# Autodesk Inventor assembly: V5H1
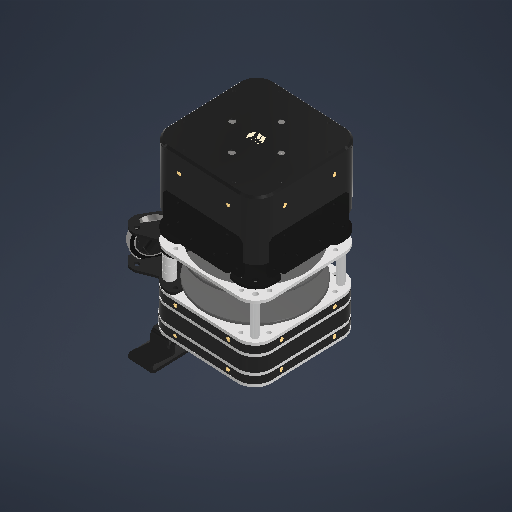
[picture p0: Inventor's stored thumbnail of the model, 512x512]
Saved by Autodesk Inventor 2026.1 (Build 301233000, 233)
## iProperties
Created: 2026-05-18
Part Number: V5H1
Document SubType Name: Assembly
Designer: aaron
Author: aaron
## Documents named in this file (18)
- D:\work\loopandpixel\openworkoutsystem\cad\v5\V5H1.iam
- D:\work\loopandpixel\openworkoutsystem\cad\v5\motor.iam
- D:\work\loopandpixel\openworkoutsystem\cad\v5\handle_metal.ipt
- D:\work\loopandpixel\openworkoutsystem\cad\v5\handle_insert.ipt
- D:\work\loopandpixel\openworkoutsystem\cad\v5\spool.iam
- D:\work\loopandpixel\openworkoutsystem\cad\v5\output_support.ipt
- D:\work\loopandpixel\openworkoutsystem\cad\v5\spool_spacer_driver.ipt
- D:\work\loopandpixel\openworkoutsystem\cad\v5\spool_spacer.ipt
- D:\work\loopandpixel\openworkoutsystem\cad\v5\M5x40mm_coupler.ipt
- D:\work\loopandpixel\openworkoutsystem\cad\v5\bearings\bearing_42x30x7.ipt
- D:\work\loopandpixel\openworkoutsystem\cad\v5\head_innter_top_42.ipt
- D:\work\loopandpixel\openworkoutsystem\cad\v5\bearings\bearing_12x8x8.ipt
- D:\work\loopandpixel\openworkoutsystem\cad\v5\stator_center_00_alu.ipt
- D:\work\loopandpixel\openworkoutsystem\cad\v5\moteus\20250427-moteus-x1-r1\20250427-moteus-x1-r1\20250427-moteus-x1-r1.ipt
- D:\work\loopandpixel\openworkoutsystem\cad\v5\20250328-x1-heat-spreader\20250328-x1-heat-spreader\20250328-x1-heat-spreader.ipt
- D:\work\loopandpixel\openworkoutsystem\cad\v5\mcthermal_plate.ipt
- D:\work\loopandpixel\openworkoutsystem\cad\v5\battery_pack_16s.ipt.iam
- battery_pack_16s.ipt
## Components (25 placed, 16 different names)
1. motor:1 [sub-assembly] — Insert:1, Insert:2, Insert:5, Insert:6, Insert:12, Insert:13
2. handle_metal:1 — Insert:1, Insert:2, Insert:3, Insert:4
3. handle_insert:1 — Insert:3, Insert:4
4. spool:1 [sub-assembly] — Insert:10, Insert:11
5. output_support:1 — Insert:16, Insert:19
6. output_support:2 — Insert:12, Insert:13, Mate:1, Insert:28, Insert:29
7. spool_spacer_driver:2 — Insert:6
8. spool_spacer_driver:3 — Insert:5, Insert:9
9. spool_spacer:1 — Insert:9, Insert:10
10. spool_spacer:2 — Insert:11
11. M5x40mm_coupler:1 — Insert:16, Insert:24, Insert:29
12. M5x40mm_coupler:2 — Insert:19, Mate:2, Insert:27, Insert:28
13. M5x40mm_coupler:3 — Insert:25
14. M5x40mm_coupler:4 — Insert:26
15. bearing_42x30x7:1 — Insert:20, Mate:1
16. head_innter_top_42:1 — Insert:20
17. bearing_12x8x8:1 — Mate:2, Insert:21
18. bearing_12x8x8:2 — Insert:21, Insert:22
19. bearing_12x8x8:3 — Insert:22, Insert:23
20. bearing_12x8x8:4 — Insert:23
21. stator_center_00_alu:1 — Insert:24, Insert:25, Insert:26, Insert:27, Flush:3, Flush:4
22. 20250427-moteus-x1-r1:1
23. 20250328-x1-heat-spreader:1
24. mcthermal_plate:1
25. battery_pack_16s.ipt:1 [sub-assembly] — Flush:3, Flush:4
## Relationships (35: Insert 27, Mate 4, Flush 4)
- Insert:1: motor:1 ↔ handle_metal:1
- Insert:2: motor:1 ↔ handle_metal:1
- Insert:3: handle_metal:1 ↔ handle_insert:1
- Insert:4: handle_metal:1 ↔ handle_insert:1
- Insert:5: motor:1 ↔ spool_spacer_driver:3
- Insert:6: motor:1 ↔ spool_spacer_driver:2
- Insert:9: spool_spacer_driver:3 ↔ spool_spacer:1
- Insert:10: spool:1 ↔ spool_spacer:1
- Insert:11: spool:1 ↔ spool_spacer:2
- Insert:12: motor:1 ↔ output_support:2
- Insert:13: motor:1 ↔ output_support:2
- Insert:16: output_support:1 ↔ M5x40mm_coupler:1
- Insert:19: output_support:1 ↔ M5x40mm_coupler:2
- Insert:20: bearing_42x30x7:1 ↔ head_innter_top_42:1
- Mate:1: output_support:2 ↔ bearing_42x30x7:1
- Mate:2: M5x40mm_coupler:2 ↔ bearing_12x8x8:1
- Insert:21: bearing_12x8x8:1 ↔ bearing_12x8x8:2
- Insert:22: bearing_12x8x8:2 ↔ bearing_12x8x8:3
- Insert:23: bearing_12x8x8:3 ↔ bearing_12x8x8:4
- Insert:24: M5x40mm_coupler:1 ↔ stator_center_00_alu:1
- Insert:25: M5x40mm_coupler:3 ↔ stator_center_00_alu:1
- Insert:26: M5x40mm_coupler:4 ↔ stator_center_00_alu:1
- Insert:27: M5x40mm_coupler:2 ↔ stator_center_00_alu:1
- Insert:28: output_support:2 ↔ M5x40mm_coupler:2
- Insert:29: output_support:2 ↔ M5x40mm_coupler:1
- [Insert]: 20250427-moteus-x1-r1:1 ↔ 20250328-x1-heat-spreader:1
- [Insert]: 20250427-moteus-x1-r1:1 ↔ 20250328-x1-heat-spreader:1
- [Mate]: 20250328-x1-heat-spreader:1 ↔ mcthermal_plate:1
- [Flush]: mcthermal_plate:1 ↔ battery_pack_16s.ipt:1
- [Flush]: mcthermal_plate:1 ↔ battery_pack_16s.ipt:1
- [Insert]: 20250328-x1-heat-spreader:1 ↔ mcthermal_plate:1
- [Insert]: 20250328-x1-heat-spreader:1 ↔ mcthermal_plate:1
- [Mate]: mcthermal_plate:1 ↔ battery_pack_16s.ipt:1
- Flush:3: stator_center_00_alu:1 ↔ battery_pack_16s.ipt:1
- Flush:4: stator_center_00_alu:1 ↔ battery_pack_16s.ipt:1
